# Autodesk Inventor assembly: LINEAR_INTAKE_ASSY
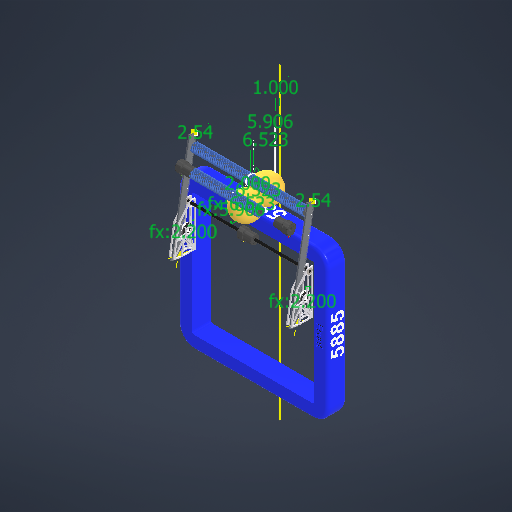
[picture p0: Inventor's stored thumbnail of the model, 512x512]
Saved by Autodesk Inventor 2026.2 (Build 302298010, 298A)
## iProperties
Created: 2026-04-01
Part Number: LINEAR_INTAKE_ASSY
Document SubType Name: Assembly
Designer: 4aida
Author: 4aida
## Documents named in this file (12)
- C:\Users\4aida\OneDrive\Documents\GitHub\2026-Robot-Mechanical\LINEAR_INTAKE\LINEAR_INTAKE_ASSY.iam
- C:\Users\4aida\OneDrive\Documents\GitHub\2026-Robot-Mechanical\Chassis\Bumpers.ipt
- C:\Users\4aida\OneDrive\Documents\GitHub\2026-Robot-Mechanical\#2_2026 Field CAD\GE-26900_ Fuel.ipt
- C:\Users\4aida\OneDrive\Documents\GitHub\2026-Robot-Mechanical\LINEAR_INTAKE\0.5_Jack_Shaft.ipt
- C:\Users\4aida\OneDrive\Documents\GitHub\2026-Robot-Mechanical\#1_CAD Library\Electronics\CONTROLS,SPARK_FLEX.ipt
- C:\Users\4aida\OneDrive\Documents\GitHub\2026-Robot-Mechanical\#1_CAD Library\Motors\MOTOR,REV,NEO,VORTEX.ipt
- C:\Users\4aida\OneDrive\Documents\GitHub\2026-Robot-Mechanical\LINEAR_INTAKE\RACK_LINEARINTAKE.ipt
- C:\Users\4aida\OneDrive\Documents\GitHub\2026-Robot-Mechanical\LINEAR_INTAKE\10DP_Pinion Gear.iam
- C:\Users\4aida\OneDrive\Documents\GitHub\2026-Robot-Mechanical\#1_CAD Library\Power Transmission\Bearings\PURCHASED,HEX_BEARING.ipt
- C:\Users\4aida\OneDrive\Documents\GitHub\2026-Robot-Mechanical\LINEAR_INTAKE\INTAKE_OUTSIDE_PLATE.ipt
- C:\Users\4aida\OneDrive\Documents\GitHub\2026-Robot-Mechanical\LINEAR_INTAKE\RACK_GUIDES.ipt
- C:\Users\4aida\OneDrive\Documents\GitHub\2026-Robot-Mechanical\LINEAR_INTAKE\CAST,2inOD,ROLLER.ipt
## Components (32 placed, 11 different names)
1. Bumpers:1 — Tangent:1, Mate:37, Mate:44, Mate:45, Tangent:3
2. 0.5_Jack_Shaft:1
3. CONTROLS,SPARK_FLEX:1
4. MOTOR,REV,NEO,VORTEX:1
5. RACK_LINEARINTAKE:1
6. 10DP_Pinion Gear:1 [sub-assembly]
7. PURCHASED,HEX_BEARING:1
8. PURCHASED,HEX_BEARING:2
9. INTAKE_OUTSIDE_PLATE:1 — Mate:44
10. INTAKE_OUTSIDE_PLATE:2
11. RACK_LINEARINTAKE:2
12. 10DP_Pinion Gear:2 [sub-assembly] — Mate:59
13. INTAKE_OUTSIDE_PLATE:3 — Mate:58, Mate:59
14. INTAKE_OUTSIDE_PLATE:4 — Mate:57
15. RACK_GUIDES:1
16. RACK_GUIDES:2 — Mate:57
17. RACK_GUIDES:3 — Mate:58
18. RACK_GUIDES:4
19. CAST,2inOD,ROLLER:1 — Mate:45, Mate:46, Mate:47
20. CAST,2inOD,ROLLER:2
21. CAST,2inOD,ROLLER:3
22. CAST,2inOD,ROLLER:4 — Flush:22
23. CAST,2inOD,ROLLER:5 — Flush:23
24. GE-26900_ Fuel:2 — Tangent:1, Tangent:2, Mate:48
25. CONTROLS,SPARK_FLEX:2 — Flush:23
26. MOTOR,REV,NEO,VORTEX:2 — Mate:49
27. CONTROLS,SPARK_FLEX:3 — Flush:22
28. MOTOR,REV,NEO,VORTEX:3 — Mate:49, Mate:55, Mate:56
29. GE-26900_ Fuel:3 — Tangent:3, Mate:50
30. CAST,2inOD,ROLLER:6 — Mate:51, Mate:52, Mate:53, Mate:54, Flush:24, Flush:25
31. CAST,2inOD,ROLLER:7 — Mate:51, Mate:54, Flush:25
32. CAST,2inOD,ROLLER:8 — Mate:52, Mate:53, Flush:24, Mate:55, Mate:56
## Relationships (84: Mate 56, Flush 25, Tangent 3)
- [Mate]: CONTROLS,SPARK_FLEX:1 ↔ MOTOR,REV,NEO,VORTEX:1
- [Mate]: CONTROLS,SPARK_FLEX:1 ↔ MOTOR,REV,NEO,VORTEX:1
- [Mate]: CONTROLS,SPARK_FLEX:1 ↔ MOTOR,REV,NEO,VORTEX:1
- [Mate]: 0.5_Jack_Shaft:1 ↔ CONTROLS,SPARK_FLEX:1
- [Mate]: 0.5_Jack_Shaft:1 ↔ MOTOR,REV,NEO,VORTEX:1
- [Mate] (30 mm): Bumpers:1 ↔ CONTROLS,SPARK_FLEX:1
- [Flush]: RACK_LINEARINTAKE:1 ↔ 10DP_Pinion Gear:1
- [Mate] (29.21 mm): RACK_LINEARINTAKE:1 ↔ 10DP_Pinion Gear:1
- [Flush]: 0.5_Jack_Shaft:1 ↔ PURCHASED,HEX_BEARING:2
- [Flush]: 0.5_Jack_Shaft:1 ↔ PURCHASED,HEX_BEARING:1
- [Mate]: 0.5_Jack_Shaft:1 ↔ PURCHASED,HEX_BEARING:1
- [Mate]: 0.5_Jack_Shaft:1 ↔ PURCHASED,HEX_BEARING:2
- [Mate]: 0.5_Jack_Shaft:1 ↔ PURCHASED,HEX_BEARING:2
- [Mate]: 0.5_Jack_Shaft:1 ↔ PURCHASED,HEX_BEARING:1
- [Mate]: PURCHASED,HEX_BEARING:2 ↔ INTAKE_OUTSIDE_PLATE:1
- [Mate]: PURCHASED,HEX_BEARING:2 ↔ INTAKE_OUTSIDE_PLATE:1
- [Flush] (6 mm): RACK_LINEARINTAKE:1 ↔ INTAKE_OUTSIDE_PLATE:1
- [Mate] (5.08 mm): RACK_LINEARINTAKE:1 ↔ INTAKE_OUTSIDE_PLATE:1
- [Mate]: PURCHASED,HEX_BEARING:1 ↔ INTAKE_OUTSIDE_PLATE:2
- [Mate]: PURCHASED,HEX_BEARING:1 ↔ INTAKE_OUTSIDE_PLATE:2
- [Flush]: RACK_LINEARINTAKE:2 ↔ 10DP_Pinion Gear:2
- [Mate] (29.21 mm): RACK_LINEARINTAKE:2 ↔ 10DP_Pinion Gear:2
- [Mate] (5.08 mm): INTAKE_OUTSIDE_PLATE:2 ↔ RACK_LINEARINTAKE:2
- [Flush]: RACK_LINEARINTAKE:1 ↔ RACK_LINEARINTAKE:2
- [Flush]: RACK_LINEARINTAKE:1 ↔ RACK_LINEARINTAKE:2
- [Mate]: 10DP_Pinion Gear:1 ↔ 10DP_Pinion Gear:2
- [Mate]: PURCHASED,HEX_BEARING:1 ↔ INTAKE_OUTSIDE_PLATE:3
- [Mate]: PURCHASED,HEX_BEARING:2 ↔ INTAKE_OUTSIDE_PLATE:4
- [Flush]: INTAKE_OUTSIDE_PLATE:1 ↔ INTAKE_OUTSIDE_PLATE:4
- [Flush]: INTAKE_OUTSIDE_PLATE:2 ↔ INTAKE_OUTSIDE_PLATE:3
- [Mate]: RACK_LINEARINTAKE:1 ↔ RACK_GUIDES:1
- [Mate]: RACK_LINEARINTAKE:2 ↔ RACK_GUIDES:3
- [Mate]: RACK_LINEARINTAKE:1 ↔ RACK_GUIDES:2
- [Mate]: RACK_LINEARINTAKE:2 ↔ RACK_GUIDES:4
- [Flush]: RACK_LINEARINTAKE:2 ↔ RACK_GUIDES:4
- [Flush]: RACK_LINEARINTAKE:2 ↔ RACK_GUIDES:4
- [Flush]: RACK_LINEARINTAKE:2 ↔ RACK_GUIDES:3
- [Flush]: RACK_LINEARINTAKE:2 ↔ RACK_GUIDES:3
- [Flush]: RACK_LINEARINTAKE:1 ↔ RACK_GUIDES:2
- [Flush]: RACK_LINEARINTAKE:1 ↔ RACK_GUIDES:2
- [Flush]: RACK_LINEARINTAKE:1 ↔ RACK_GUIDES:1
- [Flush]: RACK_LINEARINTAKE:1 ↔ RACK_GUIDES:1
- [Flush]: INTAKE_OUTSIDE_PLATE:2 ↔ RACK_GUIDES:4
- [Mate]: CAST,2inOD,ROLLER:1 ↔ CAST,2inOD,ROLLER:2
- [Mate]: CAST,2inOD,ROLLER:1 ↔ CAST,2inOD,ROLLER:3
- [Mate]: CAST,2inOD,ROLLER:2 ↔ CAST,2inOD,ROLLER:4
- [Mate]: CAST,2inOD,ROLLER:1 ↔ CAST,2inOD,ROLLER:2
- [Mate]: CAST,2inOD,ROLLER:1 ↔ CAST,2inOD,ROLLER:3
- [Mate]: CAST,2inOD,ROLLER:2 ↔ CAST,2inOD,ROLLER:4
- [Flush]: CAST,2inOD,ROLLER:2 ↔ CAST,2inOD,ROLLER:4
- [Flush]: CAST,2inOD,ROLLER:1 ↔ CAST,2inOD,ROLLER:2
- [Flush]: CAST,2inOD,ROLLER:1 ↔ CAST,2inOD,ROLLER:3
- [Mate]: CAST,2inOD,ROLLER:3 ↔ CAST,2inOD,ROLLER:5
- [Mate]: CAST,2inOD,ROLLER:3 ↔ CAST,2inOD,ROLLER:5
- Tangent:1: Bumpers:1 ↔ GE-26900_ Fuel:2
- Tangent:2: GE-26900_ Fuel:2
- Mate:37 (43.815 mm): Bumpers:1
- [Mate]: CONTROLS,SPARK_FLEX:2 ↔ MOTOR,REV,NEO,VORTEX:2
- [Mate]: CONTROLS,SPARK_FLEX:2 ↔ MOTOR,REV,NEO,VORTEX:2
- [Mate]: CONTROLS,SPARK_FLEX:2 ↔ MOTOR,REV,NEO,VORTEX:2
- [Mate]: CONTROLS,SPARK_FLEX:3 ↔ MOTOR,REV,NEO,VORTEX:3
- [Mate]: CONTROLS,SPARK_FLEX:3 ↔ MOTOR,REV,NEO,VORTEX:3
- [Mate]: CONTROLS,SPARK_FLEX:3 ↔ MOTOR,REV,NEO,VORTEX:3
- Mate:44: Bumpers:1 ↔ INTAKE_OUTSIDE_PLATE:1
- Mate:45 (165.6842 mm): Bumpers:1 ↔ CAST,2inOD,ROLLER:1
- Mate:46 (165.6842 mm): CAST,2inOD,ROLLER:1
- Mate:47: CAST,2inOD,ROLLER:1
- Mate:48: GE-26900_ Fuel:2
- Flush:22: CAST,2inOD,ROLLER:4 ↔ CONTROLS,SPARK_FLEX:3
- Flush:23: CAST,2inOD,ROLLER:5 ↔ CONTROLS,SPARK_FLEX:2
- Mate:49: MOTOR,REV,NEO,VORTEX:2 ↔ MOTOR,REV,NEO,VORTEX:3
- Tangent:3: Bumpers:1 ↔ GE-26900_ Fuel:3
- Mate:50: GE-26900_ Fuel:3
- Mate:51: CAST,2inOD,ROLLER:6 ↔ CAST,2inOD,ROLLER:7
- Mate:52: CAST,2inOD,ROLLER:6 ↔ CAST,2inOD,ROLLER:8
- Mate:53: CAST,2inOD,ROLLER:6 ↔ CAST,2inOD,ROLLER:8
- Mate:54: CAST,2inOD,ROLLER:6 ↔ CAST,2inOD,ROLLER:7
- Flush:24: CAST,2inOD,ROLLER:6 ↔ CAST,2inOD,ROLLER:8
- Flush:25: CAST,2inOD,ROLLER:6 ↔ CAST,2inOD,ROLLER:7
- Mate:55: MOTOR,REV,NEO,VORTEX:3 ↔ CAST,2inOD,ROLLER:8
- Mate:56: MOTOR,REV,NEO,VORTEX:3 ↔ CAST,2inOD,ROLLER:8
- Mate:57 (4.8387 mm): INTAKE_OUTSIDE_PLATE:4 ↔ RACK_GUIDES:2
- Mate:58 (4.8387 mm): INTAKE_OUTSIDE_PLATE:3 ↔ RACK_GUIDES:3
- Mate:59: 10DP_Pinion Gear:2 ↔ INTAKE_OUTSIDE_PLATE:3
## Named parameters: d192_d176 = 29.21 mm, d193_d174 = 0 mm, d163_d8 = 0 mm, d164_d9 = 0 mm, d165_d10 = 0 mm, d72_d163_d8 = 0 mm, d73_d164_d9 = 0 mm, d74_d165_d10 = 0 mm, d75_d163_d8 = 0 mm, d76_d164_d9 = 0 mm, d77_d165_d10 = 0 mm
